# Autodesk Inventor assembly: Ebox_assy
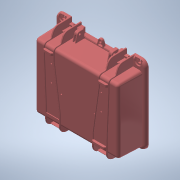
[picture p0: Inventor's stored thumbnail of the model, 180x180]
Saved by Autodesk Inventor 2021 (Build 250183000, 183)
## iProperties
Created: 2021-02-08
Part Number: Ebox_assy
Document SubType Name: Assembly
Designer: Jorian Brusind
Author: Jorian Brusind
## Documents named in this file (6)
- C:\Users\Jorian Bruslind\Documents\GitHub\PersonalProjects\HyperRail\Inventor Files\Ebox_assy.iam
- C:\Users\Jorian Bruslind\Documents\GitHub\PersonalProjects\HyperRail\Inventor Files\se300-t-b.iam
- C:\Users\Jorian Bruslind\Documents\GitHub\PersonalProjects\Inventor Projects\S-201-24.ipt
- C:\Users\Jorian Bruslind\Documents\GitHub\PersonalProjects\Inventor Projects\Useful models\Raspberry Pi 3.iam
- C:\Users\Jorian Bruslind\Documents\GitHub\PersonalProjects\HyperRail\PCB Files\ESP32 GRBL Controller\ExportSTEP\Main.iam
- C:\Users\Jorian Bruslind\Documents\GitHub\ECE44x_Senior_Design\Mechanical\Project Model Files\Inventor Files\Digikey Files\IEC320_C14_Plug\IEC320-C14.iam
## Components (5 placed, 5 different names)
1. se300-t-b:1 [sub-assembly] — Mate:9, Mate:10, Mate:11, Mate:21
2. S-201-24:1 — Mate:9, Mate:10, Mate:11, Mate:18, Mate:20, Flush:4, Flush:5, Flush:6, Flush:7, Mate:22, Mate:23
3. Raspberry Pi 3:1 [sub-assembly] — Mate:18, Flush:5, Flush:6
4. Main:1 [sub-assembly] — Mate:20, Mate:21, Flush:4
5. IEC320-C14:1 [sub-assembly] — Flush:7, Mate:22, Mate:23
## Relationships (12: Mate 8, Flush 4)
- Mate:9 (5 mm): se300-t-b:1 ↔ S-201-24:1
- Mate:10: se300-t-b:1 ↔ S-201-24:1
- Mate:11 (5 mm): se300-t-b:1 ↔ S-201-24:1
- Mate:18 (5 mm): S-201-24:1 ↔ Raspberry Pi 3:1
- Mate:20: S-201-24:1 ↔ Main:1
- Mate:21 (30 mm): se300-t-b:1 ↔ Main:1
- Flush:4 (30 mm): S-201-24:1 ↔ Main:1
- Flush:5: S-201-24:1 ↔ Raspberry Pi 3:1
- Flush:6: S-201-24:1 ↔ Raspberry Pi 3:1
- Flush:7: S-201-24:1 ↔ IEC320-C14:1
- Mate:22 (26 mm): S-201-24:1 ↔ IEC320-C14:1
- Mate:23: S-201-24:1 ↔ IEC320-C14:1
